# Autodesk Inventor assembly: RSX Assembly
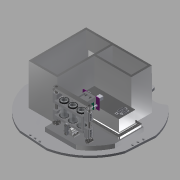
[picture p0: Inventor's stored thumbnail of the model, 180x180]
Saved by Autodesk Inventor 2017 (Build 210142000, 142)
## iProperties
Created: 2016-10-28
Part Number: RSX Assembly
Document SubType Name: Assembly
Designer: eschr_000
Author: eschr_000
## Documents named in this file (5)
- C:\Users\qupec\Desktop\UMD Near Space\STAR\CAD\Mechanical\CapTech\RSX Assembly.iam
- C:\Users\qupec\Desktop\UMD Near Space\STAR\CAD\Mechanical\CapTech\RSX Structure.ipt
- C:\Users\qupec\Desktop\UMD Near Space\STAR\CAD\Mechanical\CapTech\Pi Zero.iam
- C:\Users\qupec\Desktop\UMD Near Space\STAR\CAD\Mechanical\CapTech\Keep Out RSX Deck.ipt
- C:\Users\qupec\Desktop\UMD Near Space\STAR\CAD\Mechanical\CapTech\RSX Deck.ipt
## Components (5 placed, 5 different names)
1. RSX Structure:1 — Mate:5, Mate:7, Mate:8, Mate:16, Mate:26, Mate:32, Mate:33, Mate:38, Mate:39, Mate:40
2. Pi Zero:1 [sub-assembly] — Mate:5, Mate:7, Mate:8, Mate:32
3. Keep Out RSX Deck:1 — Mate:16
4. RSX Deck:1 — Mate:26, Mate:33, Mate:38, Mate:41
5. Full payload assembly mk 2:1 [sub-assembly] — Mate:39, Mate:40, Mate:41
## Relationships (11: Mate 11)
- Mate:5: RSX Structure:1 ↔ Pi Zero:1
- Mate:7: RSX Structure:1 ↔ Pi Zero:1
- Mate:8: RSX Structure:1 ↔ Pi Zero:1
- Mate:16: RSX Structure:1 ↔ Keep Out RSX Deck:1
- Mate:26: RSX Structure:1 ↔ RSX Deck:1
- Mate:32: RSX Structure:1 ↔ Pi Zero:1
- Mate:33: RSX Structure:1 ↔ RSX Deck:1
- Mate:38: RSX Structure:1 ↔ RSX Deck:1
- Mate:39: RSX Structure:1 ↔ Full payload assembly mk 2:1
- Mate:40: RSX Structure:1 ↔ Full payload assembly mk 2:1
- Mate:41: RSX Deck:1 ↔ Full payload assembly mk 2:1
